# Autodesk Inventor assembly: rotarynozzle
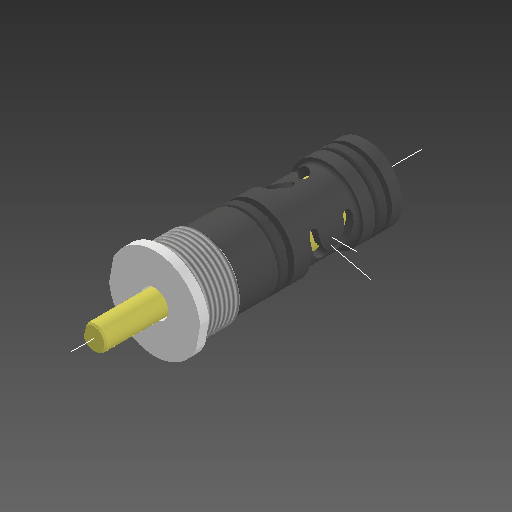
[picture p0: Inventor's stored thumbnail of the model, 512x512]
Saved by Autodesk Inventor 2021 (Build 250183000, 183)
## iProperties
Created: 2024-02-18
Part Number: rotarynozzle
Document SubType Name: Assembly
Designer: top10
Author: top10
## Documents named in this file (7)
- D:\Files\Graduation Project\V4_manfoulid\Workspaces\Workspace\R_nozzle\rotarynozzle.iam
- D:\Files\Graduation Project\V4_manfoulid\Workspaces\Workspace\R_nozzle\iner_sleeve.ipt
- D:\Files\Graduation Project\V4_manfoulid\Workspaces\Workspace\R_nozzle\outer_sleeve.ipt
- D:\Files\Graduation Project\V4_manfoulid\Workspaces\Workspace\R_nozzle\endcap.ipt
- D:\Files\Graduation Project\V4_manfoulid\Workspaces\Workspace\R_nozzle\bearing494.ipt
- D:\Files\Graduation Project\V4_manfoulid\Libraries\Content Center Files\en-US\DIN 3771(03)\DIN 3771 - 8.76 x 1.8 - N - NBR 70(4)11.88.ipt
- D:\Files\Graduation Project\V4_manfoulid\Libraries\Content Center Files\en-US\DIN 3771(06)\DIN 3771 - 4 x 1.8 - N - NBR 70(7)6.88.ipt
## Components (8 placed, 6 different names)
1. outer_sleeve:1 — Mate:1, Mate:2, Mate:5, Mate:8, Mate:10, Angle:1, Mate:11, Mate:12
2. iner_sleeve:1 — Mate:2, Mate:3, Mate:4, Mate:9, Mate:10, Angle:1, Mate:13, Mate:14
3. endcap:1 — Mate:3, Mate:8
4. bearing494:1 — Mate:4, Mate:5, Mate:9
5. DIN 3771 hydraulic (External) 8.76 x 1.8 - N - NBR 70:1 — Mate:11
6. DIN 3771 hydraulic (External) 8.76 x 1.8 - N - NBR 70:2 — Mate:12
7. DIN 3771 hydraulic and pneumatic static 4 x 1.8 - N - NBR 70:1 — Mate:13
8. DIN 3771 hydraulic and pneumatic static 4 x 1.8 - N - NBR 70:2 — Mate:14
## Relationships (13: Mate 12, Angle 1)
- Mate:1: outer_sleeve:1
- Mate:2: outer_sleeve:1 ↔ iner_sleeve:1
- Mate:3: iner_sleeve:1 ↔ endcap:1
- Mate:4: iner_sleeve:1 ↔ bearing494:1
- Mate:5: outer_sleeve:1 ↔ bearing494:1
- Mate:8: outer_sleeve:1 ↔ endcap:1
- Mate:9: iner_sleeve:1 ↔ bearing494:1
- Mate:10: outer_sleeve:1 ↔ iner_sleeve:1
- Angle:1 (-10 deg): outer_sleeve:1 ↔ iner_sleeve:1
- Mate:11: outer_sleeve:1 ↔ DIN 3771 hydraulic (External) 8.76 x 1.8 - N - NBR 70:1
- Mate:12: outer_sleeve:1 ↔ DIN 3771 hydraulic (External) 8.76 x 1.8 - N - NBR 70:2
- Mate:13: iner_sleeve:1 ↔ DIN 3771 hydraulic and pneumatic static 4 x 1.8 - N - NBR 70:1
- Mate:14: iner_sleeve:1 ↔ DIN 3771 hydraulic and pneumatic static 4 x 1.8 - N - NBR 70:2
